# Autodesk Inventor assembly: Ensamble_Balancin
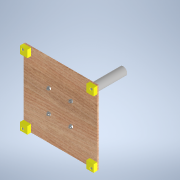
[picture p0: Inventor's stored thumbnail of the model, 180x180]
Saved by Autodesk Inventor 2022 (Build 260153000, 153)
## iProperties
Created: 2022-03-06
Part Number: Ensamble_Balancin
Document SubType Name: Assembly
Designer: hurta
Author: hurta
## Documents named in this file (10)
- C:\Users\hurta\Documents\Universidad\NovenoSemestre\MiniProyecto1\MiniProyecto1\Diseno_Mecanico_Inventor\Ensamble_Balancin.iam
- C:\Users\hurta\Documents\Universidad\NovenoSemestre\MiniProyecto1\MiniProyecto1\Diseno_Mecanico_Inventor\Base_Balancin.ipt
- C:\Users\hurta\Documents\Universidad\NovenoSemestre\MiniProyecto1\MiniProyecto1\Diseno_Mecanico_Inventor\Espaciador_Base_Balancin.ipt
- C:\Users\hurta\Documents\Universidad\NovenoSemestre\MiniProyecto1\MiniProyecto1\Diseno_Mecanico_Inventor\libreria\en-US\AS 1110\AS 1110 - M4 x 20.ipt
- C:\Users\hurta\Documents\Universidad\NovenoSemestre\MiniProyecto1\MiniProyecto1\Diseno_Mecanico_Inventor\libreria\en-US\AS 1112 (4)\AS 1112 - M4(2).ipt
- C:\Users\hurta\Documents\Universidad\NovenoSemestre\MiniProyecto1\MiniProyecto1\Diseno_Mecanico_Inventor\Union_Base_Soporte_Superior.ipt
- C:\Users\hurta\Documents\Universidad\NovenoSemestre\MiniProyecto1\MiniProyecto1\Diseno_Mecanico_Inventor\Tubo_Vertical_Soporte_Balancin.ipt
- C:\Users\hurta\Documents\Universidad\NovenoSemestre\MiniProyecto1\MiniProyecto1\Diseno_Mecanico_Inventor\libreria\en-US\AS 1112 (4)\AS 1112 - M8(2).ipt
- C:\Users\hurta\Documents\Universidad\NovenoSemestre\MiniProyecto1\MiniProyecto1\Diseno_Mecanico_Inventor\libreria\en-US\AS 1110\AS 1110 - M8 x 20.ipt
- C:\Users\hurta\Documents\Universidad\NovenoSemestre\MiniProyecto1\MiniProyecto1\Diseno_Mecanico_Inventor\libreria\en-US\AS 1111\AS 1111 - M8 x 60.ipt
## Components (25 placed, 9 different names)
1. Base_Balancin:1 — Mate:1, Mate:2, Mate:3, Mate:4, Flush:1, Flush:2, Flush:3, Flush:4, Mate:5, Mate:6, Mate:7, Mate:8, Mate:21, Mate:22, Mate:23, Mate:24, Mate:25, Mate:26, Mate:27, Mate:29, Mate:40
2. Espaciador_Base_Balancin:1 — Mate:4, Flush:3, Mate:6, Mate:12, Mate:16
3. Espaciador_Base_Balancin:2 — Mate:1, Flush:4, Mate:5, Mate:11, Mate:13
4. Espaciador_Base_Balancin:3 — Mate:3, Flush:2, Mate:8, Mate:9, Mate:15
5. Espaciador_Base_Balancin:4 — Mate:2, Flush:1, Mate:7, Mate:10, Mate:14
6. AS 1110 - Metric M4 x 20:1 — Mate:12, Mate:16, Mate:17
7. AS 1110 - Metric M4 x 20:2 — Mate:11, Mate:13, Mate:18
8. AS 1110 - Metric M4 x 20:3 — Mate:10, Mate:14, Mate:19
9. AS 1110 - Metric M4 x 20:4 — Mate:9, Mate:15, Mate:20
10. AS 1112 (4) - Metric M4:1 — Mate:19, Mate:23
11. AS 1112 (4) - Metric M4:2 — Mate:20, Mate:24
12. AS 1112 (4) - Metric M4:3 — Mate:17, Mate:22
13. AS 1112 (4) - Metric M4:4 — Mate:18, Mate:21
14. Union_Base_Soporte_Superior:1 — Mate:25, Mate:26, Mate:27, Mate:28, Mate:30, Mate:32, Mate:33, Mate:34, Mate:35, Mate:36, Mate:37, Mate:38, Mate:39
15. Tubo_Vertical_Soporte_Balancin:1 — Mate:28, Mate:29
16. AS 1112 (4) - Metric M8:1 — Mate:31
17. AS 1111 - Metric M8 x 60:1 — Mate:30, Mate:31
18. AS 1110 - Metric M8 x 20:1 — Mate:33, Mate:39, Mate:41
19. AS 1110 - Metric M8 x 20:2 — Mate:34, Mate:38, Mate:43
20. AS 1110 - Metric M8 x 20:3 — Mate:35, Mate:37, Mate:44
21. AS 1110 - Metric M8 x 20:4 — Mate:32, Mate:36, Mate:42
22. AS 1112 (4) - Metric M8:2 — Flush:5, Mate:43
23. AS 1112 (4) - Metric M8:3 — Flush:5, Flush:6, Mate:42
24. AS 1112 (4) - Metric M8:4 — Flush:6, Flush:7, Mate:40, Mate:44
25. AS 1112 (4) - Metric M8:5 — Flush:7, Mate:41
## Relationships (51: Mate 44, Flush 7)
- Mate:1: Base_Balancin:1 ↔ Espaciador_Base_Balancin:2
- Mate:2: Base_Balancin:1 ↔ Espaciador_Base_Balancin:4
- Mate:3: Base_Balancin:1 ↔ Espaciador_Base_Balancin:3
- Mate:4: Base_Balancin:1 ↔ Espaciador_Base_Balancin:1
- Flush:1: Base_Balancin:1 ↔ Espaciador_Base_Balancin:4
- Flush:2: Base_Balancin:1 ↔ Espaciador_Base_Balancin:3
- Flush:3: Base_Balancin:1 ↔ Espaciador_Base_Balancin:1
- Flush:4: Base_Balancin:1 ↔ Espaciador_Base_Balancin:2
- Mate:5: Base_Balancin:1 ↔ Espaciador_Base_Balancin:2
- Mate:6: Base_Balancin:1 ↔ Espaciador_Base_Balancin:1
- Mate:7: Base_Balancin:1 ↔ Espaciador_Base_Balancin:4
- Mate:8: Base_Balancin:1 ↔ Espaciador_Base_Balancin:3
- Mate:9: Espaciador_Base_Balancin:3 ↔ AS 1110 - Metric M4 x 20:4
- Mate:10: Espaciador_Base_Balancin:4 ↔ AS 1110 - Metric M4 x 20:3
- Mate:11: Espaciador_Base_Balancin:2 ↔ AS 1110 - Metric M4 x 20:2
- Mate:12: Espaciador_Base_Balancin:1 ↔ AS 1110 - Metric M4 x 20:1
- Mate:13: Espaciador_Base_Balancin:2 ↔ AS 1110 - Metric M4 x 20:2
- Mate:14: Espaciador_Base_Balancin:4 ↔ AS 1110 - Metric M4 x 20:3
- Mate:15: Espaciador_Base_Balancin:3 ↔ AS 1110 - Metric M4 x 20:4
- Mate:16: Espaciador_Base_Balancin:1 ↔ AS 1110 - Metric M4 x 20:1
- Mate:17: AS 1110 - Metric M4 x 20:1 ↔ AS 1112 (4) - Metric M4:3
- Mate:18: AS 1110 - Metric M4 x 20:2 ↔ AS 1112 (4) - Metric M4:4
- Mate:19: AS 1110 - Metric M4 x 20:3 ↔ AS 1112 (4) - Metric M4:1
- Mate:20: AS 1110 - Metric M4 x 20:4 ↔ AS 1112 (4) - Metric M4:2
- Mate:21: Base_Balancin:1 ↔ AS 1112 (4) - Metric M4:4
- Mate:22: Base_Balancin:1 ↔ AS 1112 (4) - Metric M4:3
- Mate:23: Base_Balancin:1 ↔ AS 1112 (4) - Metric M4:1
- Mate:24: Base_Balancin:1 ↔ AS 1112 (4) - Metric M4:2
- Mate:25: Base_Balancin:1 ↔ Union_Base_Soporte_Superior:1
- Mate:26: Base_Balancin:1 ↔ Union_Base_Soporte_Superior:1
- Mate:27: Base_Balancin:1 ↔ Union_Base_Soporte_Superior:1
- Mate:28: Union_Base_Soporte_Superior:1 ↔ Tubo_Vertical_Soporte_Balancin:1
- Mate:29: Base_Balancin:1 ↔ Tubo_Vertical_Soporte_Balancin:1
- Mate:30: Union_Base_Soporte_Superior:1 ↔ AS 1111 - Metric M8 x 60:1
- Mate:31: AS 1112 (4) - Metric M8:1 ↔ AS 1111 - Metric M8 x 60:1
- Mate:32: Union_Base_Soporte_Superior:1 ↔ AS 1110 - Metric M8 x 20:4
- Mate:33: Union_Base_Soporte_Superior:1 ↔ AS 1110 - Metric M8 x 20:1
- Mate:34: Union_Base_Soporte_Superior:1 ↔ AS 1110 - Metric M8 x 20:2
- Mate:35: Union_Base_Soporte_Superior:1 ↔ AS 1110 - Metric M8 x 20:3
- Mate:36: Union_Base_Soporte_Superior:1 ↔ AS 1110 - Metric M8 x 20:4
- Mate:37: Union_Base_Soporte_Superior:1 ↔ AS 1110 - Metric M8 x 20:3
- Mate:38: Union_Base_Soporte_Superior:1 ↔ AS 1110 - Metric M8 x 20:2
- Mate:39: Union_Base_Soporte_Superior:1 ↔ AS 1110 - Metric M8 x 20:1
- Flush:5: AS 1112 (4) - Metric M8:2 ↔ AS 1112 (4) - Metric M8:3
- Flush:6: AS 1112 (4) - Metric M8:3 ↔ AS 1112 (4) - Metric M8:4
- Flush:7: AS 1112 (4) - Metric M8:4 ↔ AS 1112 (4) - Metric M8:5
- Mate:40: Base_Balancin:1 ↔ AS 1112 (4) - Metric M8:4
- Mate:41: AS 1110 - Metric M8 x 20:1 ↔ AS 1112 (4) - Metric M8:5
- Mate:42: AS 1110 - Metric M8 x 20:4 ↔ AS 1112 (4) - Metric M8:3
- Mate:43: AS 1110 - Metric M8 x 20:2 ↔ AS 1112 (4) - Metric M8:2
- Mate:44: AS 1110 - Metric M8 x 20:3 ↔ AS 1112 (4) - Metric M8:4
